# Autodesk Inventor assembly: Rb oven housing
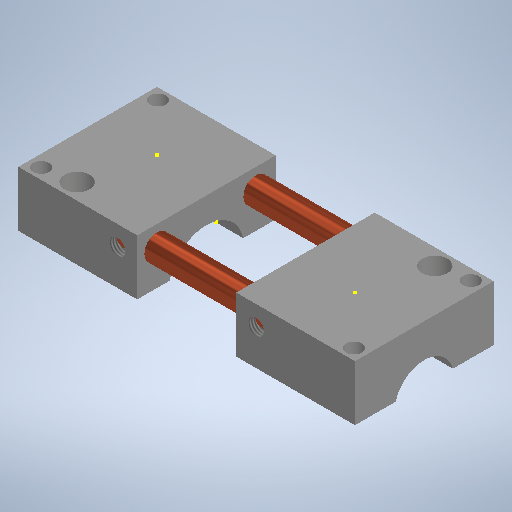
[picture p0: Inventor's stored thumbnail of the model, 512x512]
Saved by Autodesk Inventor 2025.1 (Build 291241000, 241)
## iProperties
Created: 2025-04-24
Part Number: Rb oven housing
Document SubType Name: Assembly
Designer: E. Moreno
Author: E. Moreno
Title: Carcasa Horno - Ensamblado
## Documents named in this file (4)
- C:\Users\dell 5810\Documents\M\GitHub\LAFriOC\Rb oven\Rb oven housing\Modificación\Rb oven housing - Top.iam
- C:\Users\dell 5810\Documents\M\GitHub\LAFriOC\Rb oven\Rb oven housing\Modificación\Rb oven housing post.ipt
- C:\Users\dell 5810\Documents\M\GitHub\LAFriOC\Rb oven\Rb oven housing\Modificación\Rb oven housing top-back_front.ipt
- C:\Users\dell 5810\Documents\M\GitHub\LAFriOC\Rb oven\Rb oven housing\Modificación\Rb oven housing top-back_front_MIR_MIR.ipt
## Components (4 placed, 3 different names)
1. Rb oven housing top-back_front:1 — Insertar:1, Insertar:2
2. Rb oven housing post:3 — Insertar:2
3. Rb oven housing post:4 — Insertar:1, Insertar:3
4. Rb oven housing top-back_front_MIR_MIR:1 — Insertar:3
## Relationships (3: Insert 3)
- Insertar:1 (-15 mm): Rb oven housing top-back_front:1 ↔ Rb oven housing post:4
- Insertar:2 (-15 mm): Rb oven housing top-back_front:1 ↔ Rb oven housing post:3
- Insertar:3 (-15 mm): Rb oven housing post:4 ↔ Rb oven housing top-back_front_MIR_MIR:1
